# Autodesk Inventor assembly: BatteryAdapter
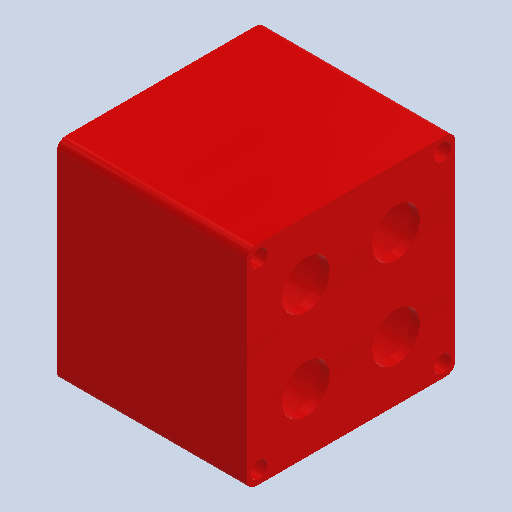
[picture p0: Inventor's stored thumbnail of the model, 512x512]
Saved by Autodesk Inventor 2022 (Build 260153000, 153)
## iProperties
Created: 2022-04-11
Part Number: BatteryAdapter
Document SubType Name: Assembly
Designer: ForseFire
Author: ForseFire
## Documents named in this file (3)
- C:\Users\Sergey\Desktop\Ariane\struct\BatteryAdapter.iam
- C:\Users\Sergey\Desktop\Ariane\struct\BatteryHolder.ipt
- C:\Users\Sergey\Desktop\Ariane\struct\BatteryRoof.ipt
## Components (2 placed, 2 different names)
1. BatteryHolder:1 — Mate:9, Flush:1, Flush:2
2. BatteryRoof:1 — Mate:9, Flush:1, Flush:2
## Relationships (3: Flush 2, Mate 1)
- Mate:9: BatteryHolder:1 ↔ BatteryRoof:1
- Flush:1: BatteryHolder:1 ↔ BatteryRoof:1
- Flush:2: BatteryHolder:1 ↔ BatteryRoof:1
